# Autodesk Inventor assembly: FALCON GEARBOX2_MIR
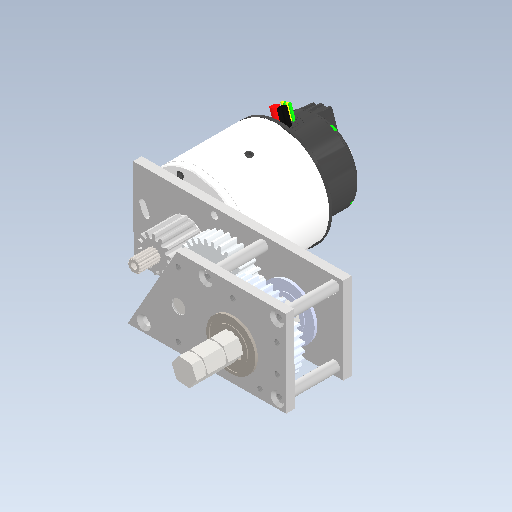
[picture p0: Inventor's stored thumbnail of the model, 512x512]
Saved by Autodesk Inventor 2021 (Build 250183000, 183)
## iProperties
Created: 2021-01-15
Part Number: FALCON GEARBOX2_MIR
Document SubType Name: Assembly
Designer: lucky
Mass: 391.615 g
Surface Area: 1131.03 cm^2
Volume: 246.948 cm^3
Density: 1.58582 g/cm^3
Author: lucky
## Documents named in this file (15)
- C:\Users\lucky\Documents\Inventor\2020DRIVEBASE\FALCON GEARBOX2_MIR.iam
- C:\Users\lucky\Documents\Inventor\2020DRIVEBASE\GEARBOX BACKPLATE_MIR.ipt
- C:\Users\lucky\Documents\Inventor\2020DRIVEBASE\GEARBOX FRONT PLATE_MIR.ipt
- C:\Users\lucky\Documents\Inventor\2020DRIVEBASE\0.5 Flanged Hex Bearing (1.125 OD) (217-3875)_MIR.ipt
- C:\Users\lucky\Documents\Inventor\2020DRIVEBASE\AIS2020\W 619_8 R-2Z_MIR.iam
- C:\Users\lucky\Documents\Inventor\2020DRIVEBASE\Falcon 500, Powered by Talon FX (217-6515)_MIR.ipt
- C:\Users\lucky\Documents\Inventor\2020DRIVEBASE\32T Aluminum Spur Gear (20 DP, 3_8_ Hex Bore) (217-5455)_MIR.ipt
- C:\Users\lucky\Documents\Inventor\2020DRIVEBASE\36T Aluminum Spur Gear (20 DP, 1_2_ Hex Bore) (217-3214)_MIR.ipt
- C:\Users\lucky\Documents\Inventor\2020DRIVEBASE\14T Aluminum Spur Gear (20 DP, 3_8_ Hex Bore) (217-2699)_MIR.ipt
- C:\Users\lucky\Documents\Inventor\2020DRIVEBASE\14T Steel Spur Gear (20 DP, Falcon Motor) (217-6922)_MIR.ipt
- C:\Users\lucky\Documents\Inventor\2020DRIVEBASE\PTO WEEK 4 TUESDAY\Workspace\WCP dual shifter\217-2731_MIR.ipt
- C:\Users\lucky\Documents\Inventor\2020DRIVEBASE\GEARBOX STANDOFFS_MIR.ipt
- C:\Users\lucky\Documents\Inventor\2020DRIVEBASE\Shaft6_MIR.ipt
- C:\Users\lucky\Documents\Inventor\2020DRIVEBASE\Shaft8_MIR.ipt
- C:\Users\lucky\Documents\Inventor\2020DRIVEBASE\BEARINGSTANDIN.ipt
## Components (18 placed, 14 different names)
1. GEARBOX BACKPLATE_MIR:1 — Mate:13, Mate:1, Mate:2, Mate:8, Mate:6, Mate:12, Mate:11, Mate:14, Mate:25, Mate:24, Mate:26, Flush:1, Mate:28, Mate:30, Mate:29, Mate:31, Mate:32, Mate:33
2. GEARBOX FRONT PLATE_MIR:1 — Mate:13, Mate:1, Mate:9, Mate:7, Mate:4, Mate:27, Mate:32
3. 0.5 Flanged Hex Bearing (1.125 OD) (217-3875)_MIR:1 — Mate:9, Mate:2, Mate:23, Angle:2
4. W 619_8 R-2Z_MIR:1 [sub-assembly] — Mate:7, Mate:4, Mate:22
5. W 619_8 R-2Z_MIR:2 [sub-assembly] — Mate:8, Mate:6, Mate:18, Mate:15, Mate:36, Mate:35
6. Falcon 500, Powered by Talon FX (217-6515)_MIR:1 — Mate:12, Mate:11, Mate:17, Mate:16
7. 32T Aluminum Spur Gear (20 DP, 3_8_ Hex Bore) (217-5455)_MIR:1 — Mate:18, Mate:15, Angle:1, Mate:21, Mate:20, Rotation:1
8. 36T Aluminum Spur Gear (20 DP, 1_2_ Hex Bore) (217-3214)_MIR:1 — Mate:23, Mate:14, Rotation:2, Angle:3
9. 14T Aluminum Spur Gear (20 DP, 3_8_ Hex Bore) (217-2699)_MIR:1 — Mate:22, Angle:1, Rotation:2, Mate:21, Mate:20, Angle:4
10. 14T Steel Spur Gear (20 DP, Falcon Motor) (217-6922)_MIR:1 — Rotation:1, Mate:17, Mate:16
11. 217-2731_MIR:1 — Mate:25, Mate:24, Mate:34, Mate:33
12. GEARBOX STANDOFFS_MIR:1 — Mate:26, Flush:1
13. GEARBOX STANDOFFS_MIR:2 — Mate:28, Mate:27
14. GEARBOX STANDOFFS_MIR:3 — Mate:30, Mate:29
15. GEARBOX STANDOFFS_MIR:4 — Mate:32, Mate:31
16. Shaft6_MIR:1 — Angle:3, Angle:2, Mate:34, Mate:33
17. Shaft8_MIR:1 — Angle:4, Mate:36, Mate:35
18. BEARINGSTANDIN:1 — Mate:32, Mate:33
## Relationships (41: Mate 33, Angle 4, RelateRotation 2, Flush 2)
- Mate:13: GEARBOX BACKPLATE_MIR:1 ↔ GEARBOX FRONT PLATE_MIR:1
- Mate:1: GEARBOX BACKPLATE_MIR:1 ↔ GEARBOX FRONT PLATE_MIR:1
- Mate:9: GEARBOX FRONT PLATE_MIR:1 ↔ 0.5 Flanged Hex Bearing (1.125 OD) (217-3875)_MIR:1
- Mate:2: GEARBOX BACKPLATE_MIR:1 ↔ 0.5 Flanged Hex Bearing (1.125 OD) (217-3875)_MIR:1
- Mate:7: GEARBOX FRONT PLATE_MIR:1 ↔ W 619_8 R-2Z_MIR:1
- Mate:4: GEARBOX FRONT PLATE_MIR:1 ↔ W 619_8 R-2Z_MIR:1
- Mate:8: GEARBOX BACKPLATE_MIR:1 ↔ W 619_8 R-2Z_MIR:2
- Mate:6: GEARBOX BACKPLATE_MIR:1 ↔ W 619_8 R-2Z_MIR:2
- Mate:12: GEARBOX BACKPLATE_MIR:1 ↔ Falcon 500, Powered by Talon FX (217-6515)_MIR:1
- Mate:11: GEARBOX BACKPLATE_MIR:1 ↔ Falcon 500, Powered by Talon FX (217-6515)_MIR:1
- Mate:18: W 619_8 R-2Z_MIR:2 ↔ 32T Aluminum Spur Gear (20 DP, 3_8_ Hex Bore) (217-5455)_MIR:1
- Mate:15: W 619_8 R-2Z_MIR:2 ↔ 32T Aluminum Spur Gear (20 DP, 3_8_ Hex Bore) (217-5455)_MIR:1
- Mate:23: 0.5 Flanged Hex Bearing (1.125 OD) (217-3875)_MIR:1 ↔ 36T Aluminum Spur Gear (20 DP, 1_2_ Hex Bore) (217-3214)_MIR:1
- Mate:14: GEARBOX BACKPLATE_MIR:1 ↔ 36T Aluminum Spur Gear (20 DP, 1_2_ Hex Bore) (217-3214)_MIR:1
- Mate:22: W 619_8 R-2Z_MIR:1 ↔ 14T Aluminum Spur Gear (20 DP, 3_8_ Hex Bore) (217-2699)_MIR:1
- Angle:1 (0 deg): 32T Aluminum Spur Gear (20 DP, 3_8_ Hex Bore) (217-5455)_MIR:1 ↔ 14T Aluminum Spur Gear (20 DP, 3_8_ Hex Bore) (217-2699)_MIR:1
- Rotation:2 [RelateRotation] (0.3889 ul): 36T Aluminum Spur Gear (20 DP, 1_2_ Hex Bore) (217-3214)_MIR:1 ↔ 14T Aluminum Spur Gear (20 DP, 3_8_ Hex Bore) (217-2699)_MIR:1
- Mate:21: 32T Aluminum Spur Gear (20 DP, 3_8_ Hex Bore) (217-5455)_MIR:1 ↔ 14T Aluminum Spur Gear (20 DP, 3_8_ Hex Bore) (217-2699)_MIR:1
- Mate:20: 32T Aluminum Spur Gear (20 DP, 3_8_ Hex Bore) (217-5455)_MIR:1 ↔ 14T Aluminum Spur Gear (20 DP, 3_8_ Hex Bore) (217-2699)_MIR:1
- Rotation:1 [RelateRotation] (0.4375 ul): 32T Aluminum Spur Gear (20 DP, 3_8_ Hex Bore) (217-5455)_MIR:1 ↔ 14T Steel Spur Gear (20 DP, Falcon Motor) (217-6922)_MIR:1
- Mate:17: Falcon 500, Powered by Talon FX (217-6515)_MIR:1 ↔ 14T Steel Spur Gear (20 DP, Falcon Motor) (217-6922)_MIR:1
- Mate:16: Falcon 500, Powered by Talon FX (217-6515)_MIR:1 ↔ 14T Steel Spur Gear (20 DP, Falcon Motor) (217-6922)_MIR:1
- Mate:25: GEARBOX BACKPLATE_MIR:1 ↔ 217-2731_MIR:1
- Mate:24: GEARBOX BACKPLATE_MIR:1 ↔ 217-2731_MIR:1
- Mate:26: GEARBOX BACKPLATE_MIR:1 ↔ GEARBOX STANDOFFS_MIR:1
- Flush:1 [Mate]: GEARBOX BACKPLATE_MIR:1 ↔ GEARBOX STANDOFFS_MIR:1
- Mate:28: GEARBOX BACKPLATE_MIR:1 ↔ GEARBOX STANDOFFS_MIR:2
- Mate:27: GEARBOX FRONT PLATE_MIR:1 ↔ GEARBOX STANDOFFS_MIR:2
- Mate:30: GEARBOX BACKPLATE_MIR:1 ↔ GEARBOX STANDOFFS_MIR:3
- Mate:29: GEARBOX BACKPLATE_MIR:1 ↔ GEARBOX STANDOFFS_MIR:3
- Mate:32: GEARBOX FRONT PLATE_MIR:1 ↔ GEARBOX STANDOFFS_MIR:4
- Mate:31: GEARBOX BACKPLATE_MIR:1 ↔ GEARBOX STANDOFFS_MIR:4
- Angle:3 (0 deg): 36T Aluminum Spur Gear (20 DP, 1_2_ Hex Bore) (217-3214)_MIR:1 ↔ Shaft6_MIR:1
- Angle:2 (0 deg): 0.5 Flanged Hex Bearing (1.125 OD) (217-3875)_MIR:1 ↔ Shaft6_MIR:1
- Mate:34 [Flush]: 217-2731_MIR:1 ↔ Shaft6_MIR:1
- Mate:33: 217-2731_MIR:1 ↔ Shaft6_MIR:1
- Angle:4 (0 deg): 14T Aluminum Spur Gear (20 DP, 3_8_ Hex Bore) (217-2699)_MIR:1 ↔ Shaft8_MIR:1
- Mate:36 [Flush]: W 619_8 R-2Z_MIR:2 ↔ Shaft8_MIR:1
- Mate:35: W 619_8 R-2Z_MIR:2 ↔ Shaft8_MIR:1
- Mate:32: GEARBOX BACKPLATE_MIR:1 ↔ BEARINGSTANDIN:1
- Mate:33: GEARBOX BACKPLATE_MIR:1 ↔ BEARINGSTANDIN:1
